# Autodesk Inventor assembly: Finished_Basement_And_First_Floor
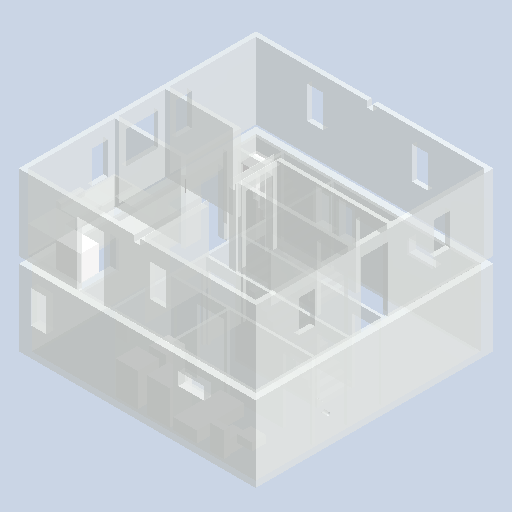
[picture p0: Inventor's stored thumbnail of the model, 512x512]
Saved by Autodesk Inventor 2024 (Build 280153020, 153B)
## iProperties
Created: 2023-05-18
Part Number: Finished_Basement_And_First_Floor
Document SubType Name: Assembly
Designer: Tom
Author: Tom
## Documents named in this file (10)
- C:\Users\Tom\Documents\Tom_Levers_Public_Git_Repository\Inventor\Mobility\Finished_Basement_And_First_Floor.iam
- C:\Users\Tom\Documents\Tom_Levers_Public_Git_Repository\Inventor\Mobility\Basement\Finished_Basement.iam
- C:\Users\Tom\Documents\Tom_Levers_Public_Git_Repository\Inventor\Mobility\First_Floor\Finished_First_Floor.iam
- C:\Users\Tom\Documents\Tom_Levers_Public_Git_Repository\Inventor\Mobility\First_Floor\Window_Cabinet\Window_Cabinet.iam
- C:\Users\Tom\Documents\Tom_Levers_Public_Git_Repository\Inventor\Mobility\First_Floor\Range.ipt
- C:\Users\Tom\Documents\Tom_Levers_Public_Git_Repository\Inventor\Mobility\First_Floor\Stairs_Between_First_Floor_And_Second_Floor.ipt
- C:\Users\Tom\Documents\Tom_Levers_Public_Git_Repository\Inventor\Mobility\Finished_Basement_And_First_Floor\AIP\FEA\eeawfczi8.fins
- C:\Users\Tom\Documents\Tom_Levers_Public_Git_Repository\Inventor\Mobility\Finished_Basement_And_First_Floor\AIP\FEA\eeawfczi8.fsat
- C:\Users\Tom\Documents\Tom_Levers_Public_Git_Repository\Inventor\Mobility\Finished_Basement_And_First_Floor\AIP\FEA\eeawfczi8.ftes
- C:\Users\Tom\Documents\Tom_Levers_Public_Git_Repository\Inventor\Mobility\Finished_Basement_And_First_Floor\AIP\FEA\eeawfczi8.fwiz
## Components (5 placed, 5 different names)
1. Finished_Basement:1 [sub-assembly] — Flush:3, Flush:4
2. Finished_First_Floor:1 [sub-assembly] — Mate:8, Mate:9, Flush:3, Flush:4
3. Window_Cabinet:1 [sub-assembly]
4. Range:1
5. Stairs_Between_First_Floor_And_Second_Floor:1 — Mate:8, Mate:9
## Relationships (4: Mate 2, Flush 2)
- Mate:8 (1244.6 mm): Finished_First_Floor:1 ↔ Stairs_Between_First_Floor_And_Second_Floor:1
- Mate:9: Finished_First_Floor:1 ↔ Stairs_Between_First_Floor_And_Second_Floor:1
- Flush:3: Finished_Basement:1 ↔ Finished_First_Floor:1
- Flush:4 (215.9 mm): Finished_Basement:1 ↔ Finished_First_Floor:1
## Named parameters: sa_0 = 980.999, sa_1 = 19.1674, sa_2 = 19.1674
note: some values were not read from the file. Shown as the stored number, unit unknown: "sa_0", "sa_1", "sa_2".
